# Autodesk Inventor assembly: ASY MSC 204 BELLY
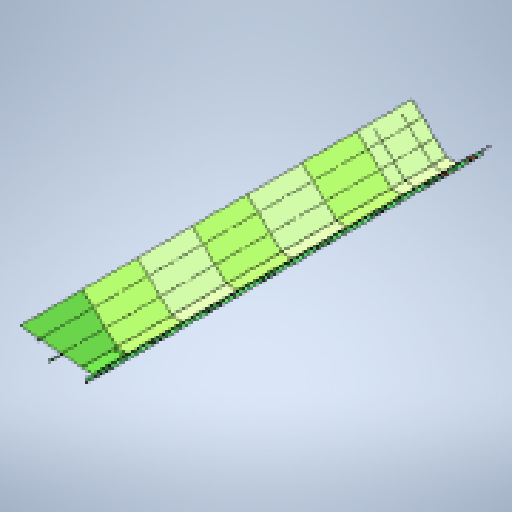
[picture p0: Inventor's stored thumbnail of the model, 512x512]
Saved by Autodesk Inventor 2025 (Build 290162010, 162A)
## iProperties
Created: 2024-07-22
Part Number: ASY MSC 204 BELLY
Document SubType Name: Assembly
Designer: pokla
Author: pokla
## Documents named in this file (5)
- C:\Users\admin\YandexDisk-badmisterfox\домашниий пк\Inventor\Manturovo\Manturovo_Se-clar\ASY MSC 204 BELLY.iam
- C:\Users\admin\YandexDisk-badmisterfox\домашниий пк\Inventor\Manturovo\Manturovo_Se-clar\MSC 041 sheet belly main.ipt
- C:\Users\admin\YandexDisk-badmisterfox\домашниий пк\Inventor\Manturovo\Manturovo_Se-clar\MSC 042 sheet belly-neck.ipt
- C:\Users\admin\YandexDisk-badmisterfox\домашниий пк\Inventor\Manturovo\Manturovo_Se-clar\MSC 067 stringer board belly.ipt
- C:\Users\admin\YandexDisk-badmisterfox\домашниий пк\Inventor\Manturovo\Manturovo_Se-clar\MSC 053 rib belly.ipt
## Components (39 placed, 5 different names)
1. MSC 041 sheet belly main.ipt:1
2. MSC 041 sheet belly main.ipt:2
3. MSC 041 sheet belly main.ipt:3
4. MSC 042 sheet belly-neck.ipt:1 — Rigid:22
5. MSC 041 sheet belly main.ipt:4
6. MSC 041 sheet belly main.ipt:5 — Rigid:22
7. MSC 041 sheet belly main.ipt:6 — Mate:4, Mate:5, Mate:6, Mate:7, Flush:1, Mate:9, Mate:10, Flush:2, Mate:11, Mate:12
8. MSC 053 rib belly.ipt:4 — Rigid:17, Rigid:20, Rigid:21, Mate:13
9. MSC 053 rib belly.ipt:3 — Rigid:18, Rigid:19, Mate:11, Mate:12, Mate:13
10. MSC 067 stringer board belly.ipt:5 — Rigid:21, Flush:2
11. MSC 067 stringer board belly.ipt:6 — Rigid:20
12. MSC 067 stringer board belly.ipt:8 — Rigid:19
13. MSC 067 stringer board belly.ipt:7 — Rigid:18
14. MSC 053 rib belly.ipt:1 — Mate:6, Mate:7, Mate:8, Rigid:17
15. MSC 053 rib belly.ipt:2 — Mate:4, Mate:5, Mate:8
16. MSC 067 stringer board belly.ipt:2
17. MSC 067 stringer board belly.ipt:1
18. MSC 067 stringer board belly.ipt:3
19. MSC 067 stringer board belly.ipt:4
20. МОО 057 стрингер борт 7:11
21. МОО 057 стрингер борт 7:12
22. МОО 057 стрингер борт 7:13
23. МОО 057 стрингер борт 7:14
24. МОО 057 стрингер борт 7:15
25. МОО 057 стрингер борт 7:16
26. МОО 057 стрингер борт 7:17
27. МОО 057 стрингер борт 7:18
28. МОО 057 стрингер борт 7:19
29. МОО 057 стрингер борт 7:20
30. МОО 057 стрингер борт 7:21
31. МОО 057 стрингер борт 7:22
32. МОО 057 стрингер борт 7:23
33. МОО 057 стрингер борт 7:24
34. МОО 057 стрингер борт 7:25
35. МОО 057 стрингер борт 7:26
36. МОО 057 стрингер борт 7:27
37. МОО 057 стрингер борт 7:28
38. МОО 057 стрингер борт 7:29
39. МОО 057 стрингер борт 7:30
## Component patterns: (6 elements, first: MSC 067 stringer board belly.ipt:2 + MSC 067 stringer board belly.ipt:1 + MSC 067 stringer board belly.ipt:3 + MSC 067 stringer board belly.ipt:4)
## Relationships (27: WeldJoint 15, Mate 10, Flush 2)
- [WeldJoint]: MSC 041 sheet belly main.ipt:1 ↔ MSC 041 sheet belly main.ipt:2
- [WeldJoint]: MSC 041 sheet belly main.ipt:1 ↔ MSC 041 sheet belly main.ipt:3
- [WeldJoint]: MSC 041 sheet belly main.ipt:4 ↔ MSC 041 sheet belly main.ipt:5
- [WeldJoint]: MSC 041 sheet belly main.ipt:3 ↔ MSC 041 sheet belly main.ipt:4
- [WeldJoint]: MSC 041 sheet belly main.ipt:2 ↔ MSC 041 sheet belly main.ipt:6
- [WeldJoint]: MSC 067 stringer board belly.ipt:8 ↔ MSC 067 stringer board belly.ipt:2
- [WeldJoint]: MSC 067 stringer board belly.ipt:7 ↔ MSC 067 stringer board belly.ipt:1
- [WeldJoint]: MSC 067 stringer board belly.ipt:6 ↔ MSC 067 stringer board belly.ipt:3
- [WeldJoint]: MSC 067 stringer board belly.ipt:5 ↔ MSC 067 stringer board belly.ipt:4
- Mate:4: MSC 041 sheet belly main.ipt:6 ↔ MSC 053 rib belly.ipt:2
- Mate:5: MSC 041 sheet belly main.ipt:6 ↔ MSC 053 rib belly.ipt:2
- Mate:6: MSC 041 sheet belly main.ipt:6 ↔ MSC 053 rib belly.ipt:1
- Mate:7: MSC 041 sheet belly main.ipt:6 ↔ MSC 053 rib belly.ipt:1
- Mate:8: MSC 053 rib belly.ipt:1 ↔ MSC 053 rib belly.ipt:2
- Flush:1: MSC 041 sheet belly main.ipt:6
- Mate:9: MSC 041 sheet belly main.ipt:6
- Mate:10: MSC 041 sheet belly main.ipt:6
- Rigid:17 [WeldJoint] (480 mm): MSC 053 rib belly.ipt:4 ↔ MSC 053 rib belly.ipt:1
- Rigid:18 [WeldJoint]: MSC 053 rib belly.ipt:3 ↔ MSC 067 stringer board belly.ipt:7
- Rigid:19 [WeldJoint]: MSC 053 rib belly.ipt:3 ↔ MSC 067 stringer board belly.ipt:8
- Rigid:20 [WeldJoint]: MSC 053 rib belly.ipt:4 ↔ MSC 067 stringer board belly.ipt:6
- Rigid:21 [WeldJoint]: MSC 053 rib belly.ipt:4 ↔ MSC 067 stringer board belly.ipt:5
- Flush:2: MSC 041 sheet belly main.ipt:6 ↔ MSC 067 stringer board belly.ipt:5
- Rigid:22 [WeldJoint]: MSC 042 sheet belly-neck.ipt:1 ↔ MSC 041 sheet belly main.ipt:5
- Mate:11: MSC 041 sheet belly main.ipt:6 ↔ MSC 053 rib belly.ipt:3
- Mate:12: MSC 041 sheet belly main.ipt:6 ↔ MSC 053 rib belly.ipt:3
- Mate:13: MSC 053 rib belly.ipt:4 ↔ MSC 053 rib belly.ipt:3
